# Autodesk Inventor assembly: BatteryArrangement1
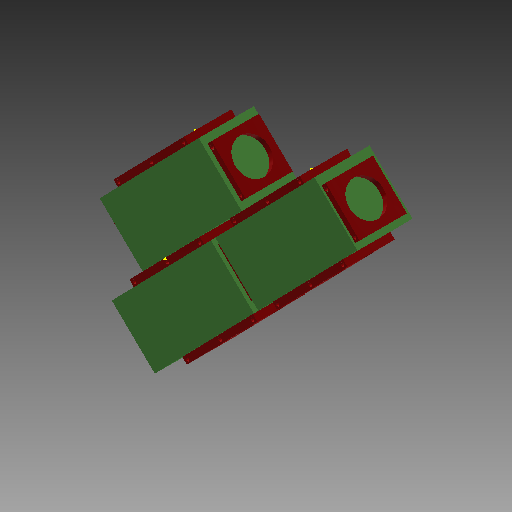
[picture p0: Inventor's stored thumbnail of the model, 512x512]
Saved by Autodesk Inventor 2019.3 (Build 233278000, 278)
## iProperties
Created: 2018-09-28
Part Number: BatteryArrangement1
Document SubType Name: Assembly
Designer: eroldan
Author: eroldan
## Documents named in this file (4)
- C:\Users\eroldan\Desktop\3dprojects\OpenEmoto\MainFrame\Battery\BatteryArrangement.iam
- C:\Users\eroldan\Desktop\3dprojects\OpenEmoto\MainFrame\Battery\Multistar-6S-16Ah.ipt
- C:\Users\eroldan\Desktop\3dprojects\OpenEmoto\MainFrame\Battery\SpacerBig.ipt
- C:\Users\eroldan\Desktop\3dprojects\OpenEmoto\MainFrame\Battery\SpacerSmall.ipt
## Components (13 placed, 3 different names)
1. SpacerBig:1 — Mate:1, Mate:3
2. Multistar-6S-16Ah:2 — Mate:1, Mate:2, Mate:6, Mate:8, Flush:2
3. Multistar-6S-16Ah:3 — Mate:3, Mate:7, Mate:13, Flush:1, Flush:3, Mate:14
4. SpacerBig:2 — Mate:2
5. SpacerSmall:2 — Mate:8
6. SpacerSmall:3 — Mate:6
7. SpacerSmall:4 — Mate:7
8. SpacerBig:4 — Mate:13
9. Multistar-6S-16Ah:4 — Flush:1, Flush:4, Mate:15, Mate:16, Mate:17, Mate:18
10. SpacerSmall:5 — Mate:14, Mate:15
11. SpacerSmall:6 — Mate:16
12. SpacerBig:5 — Mate:17
13. SpacerBig:6 — Mate:18
## Relationships (16: Mate 12, Flush 4)
- Mate:1: SpacerBig:1 ↔ Multistar-6S-16Ah:2
- Mate:2: Multistar-6S-16Ah:2 ↔ SpacerBig:2
- Mate:3: SpacerBig:1 ↔ Multistar-6S-16Ah:3
- Mate:6: Multistar-6S-16Ah:2 ↔ SpacerSmall:3
- Mate:7: Multistar-6S-16Ah:3 ↔ SpacerSmall:4
- Mate:8: Multistar-6S-16Ah:2 ↔ SpacerSmall:2
- Mate:13: Multistar-6S-16Ah:3 ↔ SpacerBig:4
- Flush:1: Multistar-6S-16Ah:3 ↔ Multistar-6S-16Ah:4
- Flush:2: Multistar-6S-16Ah:2
- Flush:3: Multistar-6S-16Ah:3
- Flush:4: Multistar-6S-16Ah:4
- Mate:14: Multistar-6S-16Ah:3 ↔ SpacerSmall:5
- Mate:15: Multistar-6S-16Ah:4 ↔ SpacerSmall:5
- Mate:16: Multistar-6S-16Ah:4 ↔ SpacerSmall:6
- Mate:17: Multistar-6S-16Ah:4 ↔ SpacerBig:5
- Mate:18: Multistar-6S-16Ah:4 ↔ SpacerBig:6
